# Autodesk Inventor assembly: Assembly1
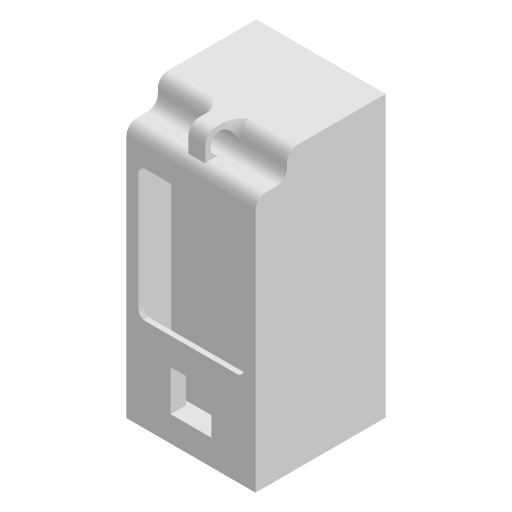
[picture p0: Inventor's stored thumbnail of the model, 512x512]
Saved by Autodesk Inventor 2023.3 (Build 273359000, 359)
## iProperties
Created: 2025-03-15
Part Number: Assembly1
Document SubType Name: Assembly
Designer: David Zindović
Author: David Zindović
## Documents named in this file (7)
- C:\Users\David Zindović\Desktop\Projekti\Darila\MyFlower\Ohisje_z_baterijo\Assembly1.iam
- C:\Users\David Zindović\Desktop\Projekti\Darila\MyFlower\Ohisje_z_baterijo\Part1.ipt
- C:\Users\David Zindović\Desktop\Projekti\Darila\MyFlower\Ohisje_z_baterijo\Part2.ipt
- C:\Users\David Zindović\Desktop\Projekti\Darila\MyFlower\Ohisje_z_baterijo\Cepek1.ipt
- C:\Users\David Zindović\Desktop\Projekti\Darila\MyFlower\Ohisje_z_baterijo\Cepek2.ipt
- C:\Users\David Zindović\Desktop\Projekti\Darila\MyFlower\Ohisje_z_baterijo\vrata.ipt
- C:\Users\David Zindović\Desktop\Projekti\Darila\MyFlower\Ohisje_z_baterijo\cepek srauf zadi.ipt
## Components (7 placed, 6 different names)
1. Part1:1 — Mate:1, Mate:2, Mate:3, Mate:4, Flush:1, Mate:5, Mate:6, Flush:2, Mate:7, Mate:8, Mate:9, Flush:3, Mate:10, Flush:4, Mate:11, Flush:5
2. Part2:1 — Mate:1, Mate:2, Mate:3
3. Cepek1:1 — Mate:4, Flush:1, Mate:5
4. Cepek2:1 — Mate:6, Flush:2, Mate:7
5. vrata:1 — Mate:8, Mate:9, Flush:3
6. cepek srauf zadi:1 — Mate:11, Flush:5
7. cepek srauf zadi:2 — Mate:10, Flush:4
## Relationships (16: Mate 11, Flush 5)
- Mate:1: Part1:1 ↔ Part2:1
- Mate:2: Part1:1 ↔ Part2:1
- Mate:3: Part1:1 ↔ Part2:1
- Mate:4: Part1:1 ↔ Cepek1:1
- Flush:1: Part1:1 ↔ Cepek1:1
- Mate:5: Part1:1 ↔ Cepek1:1
- Mate:6: Part1:1 ↔ Cepek2:1
- Flush:2: Part1:1 ↔ Cepek2:1
- Mate:7: Part1:1 ↔ Cepek2:1
- Mate:8: Part1:1 ↔ vrata:1
- Mate:9: Part1:1 ↔ vrata:1
- Flush:3: Part1:1 ↔ vrata:1
- Mate:10: Part1:1 ↔ cepek srauf zadi:2
- Flush:4: Part1:1 ↔ cepek srauf zadi:2
- Mate:11: Part1:1 ↔ cepek srauf zadi:1
- Flush:5: Part1:1 ↔ cepek srauf zadi:1
